# Autodesk Inventor assembly: Screen assembly
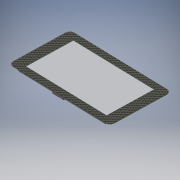
[picture p0: Inventor's stored thumbnail of the model, 180x180]
Saved by Autodesk Inventor 2017 SP1 (Build 210196100, 196)
## iProperties
Part Number: Screen assembly
Material: Generisch
Document SubType Name: Assembly
Designer: u26048
Author: u26048
## Documents named in this file (7)
- C:\Users\Stanley\Documents\Inventor\Projects\3D-Printer\3D_Printer_Parts\Selfmade_Parts\Raspberrypi 7inch display\Screen assembly.iam
- C:\Users\Stanley\Documents\Inventor\Projects\3D-Printer\3D_Printer_Parts\Selfmade_Parts\Raspberrypi 7inch display\Display Lens.ipt
- C:\Users\Stanley\Documents\Inventor\Projects\3D-Printer\3D_Printer_Parts\Selfmade_Parts\Raspberrypi 7inch display\Display Glass.ipt
- C:\Users\Stanley\Documents\Inventor\Projects\3D-Printer\3D_Printer_Parts\Selfmade_Parts\Raspberrypi 7inch display\Display Controller.ipt
- C:\Users\Stanley\Documents\Inventor\Projects\3D-Printer\3D_Printer_Parts\Selfmade_Parts\Raspberrypi 7inch display\Pi Foundation Display Driver Board.ipt
- C:\Users\Stanley\Documents\Inventor\Projects\3D-Printer\3D_Printer_Parts\Selfmade_Parts\Raspberrypi 7inch display\Spacer.ipt
- C:\Users\Stanley\Documents\Inventor\Projects\3D-Printer\3D_Printer_Parts\Selfmade_Parts\Raspberrypi3\Raspberry Pi 3.iam
## Components (9 placed, 6 different names)
1. Display Lens:1 — Fluchtend:1, Passend:1, Passend:2, Passend:3, Fluchtend:2, Fluchtend:3
2. Display Glass:1 — Fluchtend:1, Passend:1, Passend:2
3. Display Controller:1 — Passend:3, Fluchtend:2, Fluchtend:3, Passend:4, Passend:6, Passend:8, Passend:20, Passend:21, Passend:22, Passend:23
4. Pi Foundation Display Driver Board:1 — Passend:4, Passend:6, Passend:7, Passend:9, Passend:11, Passend:13, Passend:21
5. Spacer:1 — Passend:7, Passend:8, Passend:15, Passend:24
6. Spacer:2 — Passend:9, Passend:22
7. Spacer:3 — Passend:13, Passend:23, Passend:25
8. Spacer:4 — Passend:11, Passend:18, Passend:20
9. Raspberry Pi 3:1 [sub-assembly] — Passend:15, Passend:18, Passend:24, Passend:25
## Relationships (21: Mate 18, Flush 3)
- Fluchtend:1 [Flush]: Display Lens:1 ↔ Display Glass:1
- Passend:1 [Mate]: Display Lens:1 ↔ Display Glass:1
- Passend:2 [Mate]: Display Lens:1 ↔ Display Glass:1
- Passend:3 [Mate]: Display Lens:1 ↔ Display Controller:1
- Fluchtend:2 [Flush] (12 mm): Display Lens:1 ↔ Display Controller:1
- Fluchtend:3 [Flush] (6.63 mm): Display Lens:1 ↔ Display Controller:1
- Passend:4 [Mate]: Display Controller:1 ↔ Pi Foundation Display Driver Board:1
- Passend:6 [Mate]: Display Controller:1 ↔ Pi Foundation Display Driver Board:1
- Passend:7 [Mate]: Pi Foundation Display Driver Board:1 ↔ Spacer:1
- Passend:8 [Mate]: Display Controller:1 ↔ Spacer:1
- Passend:9 [Mate]: Pi Foundation Display Driver Board:1 ↔ Spacer:2
- Passend:11 [Mate]: Pi Foundation Display Driver Board:1 ↔ Spacer:4
- Passend:13 [Mate]: Pi Foundation Display Driver Board:1 ↔ Spacer:3
- Passend:15 [Mate]: Spacer:1 ↔ Raspberry Pi 3:1
- Passend:18 [Mate]: Spacer:4 ↔ Raspberry Pi 3:1
- Passend:20 [Mate]: Display Controller:1 ↔ Spacer:4
- Passend:21 [Mate]: Display Controller:1 ↔ Pi Foundation Display Driver Board:1
- Passend:22 [Mate]: Display Controller:1 ↔ Spacer:2
- Passend:23 [Mate]: Display Controller:1 ↔ Spacer:3
- Passend:24 [Mate]: Spacer:1 ↔ Raspberry Pi 3:1
- Passend:25 [Mate]: Spacer:3 ↔ Raspberry Pi 3:1
